# Autodesk Inventor assembly: A_openmechanism
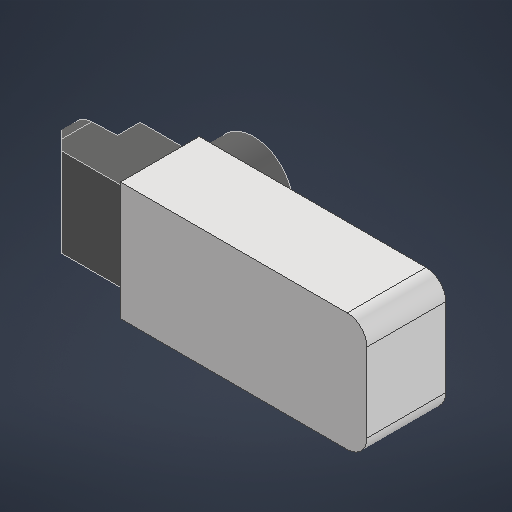
[picture p0: Inventor's stored thumbnail of the model, 512x512]
Saved by Autodesk Inventor 2026.2 (Build 302298000, 298)
## iProperties
Created: 2025-09-04
Part Number: A_openmechanism
Document SubType Name: Assembly
Designer: FAL
Author: FAL
## Documents named in this file (3)
- C:\Users\FAL\git\AIRBERT\CAD\Fuselage\openmechanism\A_openmechanism.iam
- C:\Users\FAL\git\AIRBERT\CAD\Fuselage\openmechanism\P_handle.ipt
- C:\Users\FAL\git\AIRBERT\CAD\Fuselage\openmechanism\P_Case.ipt
## Components (2 placed, 2 different names)
1. P_handle:1 — Fluchtend:7, Passend:1, Passend:2
2. P_Case:1 — Fluchtend:1, Fluchtend:2, Fluchtend:3, Passend:1, Passend:2
## Relationships (6: Flush 4, Mate 2)
- Fluchtend:1 [Flush]: P_Case:1
- Fluchtend:2 [Flush]: P_Case:1
- Fluchtend:3 [Flush]: P_Case:1
- Fluchtend:7 [Flush]: P_handle:1
- Passend:1 [Mate]: P_handle:1 ↔ P_Case:1
- Passend:2 [Mate] (14 mm): P_handle:1 ↔ P_Case:1
